# Autodesk Inventor assembly: przekladnia
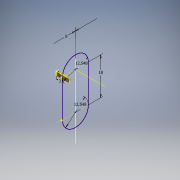
[picture p0: Inventor's stored thumbnail of the model, 180x180]
Saved by Autodesk Inventor 2019 (Build 230136000, 136)
## iProperties
Created: 2020-05-17
Part Number: przekladnia
Document SubType Name: Assembly
Designer: estee
Author: estee
## Documents named in this file (3)
- C:\Users\estee\OneDrive\Pulpit\estere\1\MUM\projejt\przekladnia.iam
- C:\Users\estee\OneDrive\Pulpit\estere\1\MUM\projejt\przekladnia.ipt
- C:\Users\estee\OneDrive\Pulpit\estere\1\MUM\projejt\zab.ipt
## Components (2 placed, 2 different names)
1. przekladnia:1 — Flush:1, Flush:2, Flush:3, Mate:1, Angle:1, Mate:2, Angle:2
2. zab:1 — Mate:1, Flush:4, Angle:1
## Relationships (8: Flush 4, Mate 2, Angle 2)
- Flush:1: przekladnia:1
- Flush:2: przekladnia:1
- Flush:3: przekladnia:1
- Mate:1: przekladnia:1 ↔ zab:1
- Flush:4 (-3 mm): zab:1
- Angle:1 (0 deg): przekladnia:1 ↔ zab:1
- Mate:2: przekladnia:1
- Angle:2 (0 deg): przekladnia:1
